# Autodesk Inventor assembly: Wind Tunnel Assembly
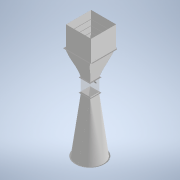
[picture p0: Inventor's stored thumbnail of the model, 180x180]
Saved by Autodesk Inventor 2022 (Build 260153000, 153)
## iProperties
Created: 2022-03-06
Part Number: Wind Tunnel Assembly
Document SubType Name: Assembly
Designer: calvi
Author: calvi
## Documents named in this file (5)
- E:\Dr. A Muchiri\Wind tunnel_Dr.A Muchiri\Wind Tunnel Assembly.iam
- E:\Dr. A Muchiri\Wind tunnel_Dr.A Muchiri\Entrance Assembly.iam
- E:\Dr. A Muchiri\Wind tunnel_Dr.A Muchiri\Contraction Assembly.iam
- E:\Dr. A Muchiri\Wind tunnel_Dr.A Muchiri\Diffuser.ipt
- E:\Dr. A Muchiri\Wind tunnel_Dr.A Muchiri\updatedtestsectionassembly.iam
## Components (4 placed, 4 different names)
1. Entrance Assembly:1 [sub-assembly] — Flush:1, Flush:2, Mate:1
2. Contraction Assembly:1 [sub-assembly] — Flush:1, Flush:2, Mate:1, Flush:3, Mate:2, Flush:4
3. updatedtestsectionassembly:1 [sub-assembly] — Flush:3, Mate:2, Flush:4, Flush:5, Mate:3
4. Diffuser:1 — Flush:5, Mate:3
## Relationships (8: Flush 5, Mate 3)
- Flush:1: Entrance Assembly:1 ↔ Contraction Assembly:1
- Flush:2: Entrance Assembly:1 ↔ Contraction Assembly:1
- Mate:1: Entrance Assembly:1 ↔ Contraction Assembly:1
- Flush:3: Contraction Assembly:1 ↔ updatedtestsectionassembly:1
- Mate:2: Contraction Assembly:1 ↔ updatedtestsectionassembly:1
- Flush:4: Contraction Assembly:1 ↔ updatedtestsectionassembly:1
- Flush:5: updatedtestsectionassembly:1 ↔ Diffuser:1
- Mate:3: updatedtestsectionassembly:1 ↔ Diffuser:1
